# Autodesk Inventor assembly: Shelf
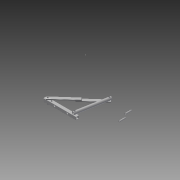
[picture p0: Inventor's stored thumbnail of the model, 180x180]
Saved by Autodesk Inventor 2013 (Build 170138000, 138)
## iProperties
Created: 2014-05-22
Part Number: Shelf
Document SubType Name: Assembly
Designer: nojessen
Author: nojessen
## Documents named in this file (6)
- C:\Users\nojessen\Documents\GitHub\IED_Virtual_Design_Challenge\CAD\Shelf.iam
- C:\Users\nojessen\Documents\GitHub\IED_Virtual_Design_Challenge\CAD\Clip for Pin.ipt
- C:\Users\nojessen\Documents\GitHub\IED_Virtual_Design_Challenge\CAD\Diagonal Supporter.ipt
- C:\Users\nojessen\Documents\GitHub\IED_Virtual_Design_Challenge\CAD\Horizantal Rod.ipt
- C:\Users\nojessen\Documents\GitHub\IED_Virtual_Design_Challenge\CAD\Pin.ipt
- C:\Users\nojessen\Documents\GitHub\IED_Virtual_Design_Challenge\CAD\Vertical Rod.ipt
## Components (7 placed, 5 different names)
1. Clip for Pin:1
2. Diagonal Supporter:1 — Mate:3, Mate:4, Mate:5, Mate:6, Mate:7
3. Horizantal Rod:1 — Mate:1, Mate:2, Mate:3
4. Vertical Rod:1 — Mate:1, Mate:2, Mate:4, Mate:5
5. Pin:1 — Mate:6, Mate:7
6. Pin:2
7. Pin:3
## Relationships (7: Mate 7)
- Mate:1: Horizantal Rod:1 ↔ Vertical Rod:1
- Mate:2 (12.7 mm): Horizantal Rod:1 ↔ Vertical Rod:1
- Mate:3: Diagonal Supporter:1 ↔ Horizantal Rod:1
- Mate:4: Diagonal Supporter:1 ↔ Vertical Rod:1
- Mate:5: Diagonal Supporter:1 ↔ Vertical Rod:1
- Mate:6: Diagonal Supporter:1 ↔ Pin:1
- Mate:7: Diagonal Supporter:1 ↔ Pin:1
